# Autodesk Inventor assembly: ITEM_41115_Winkelsatz_90deg
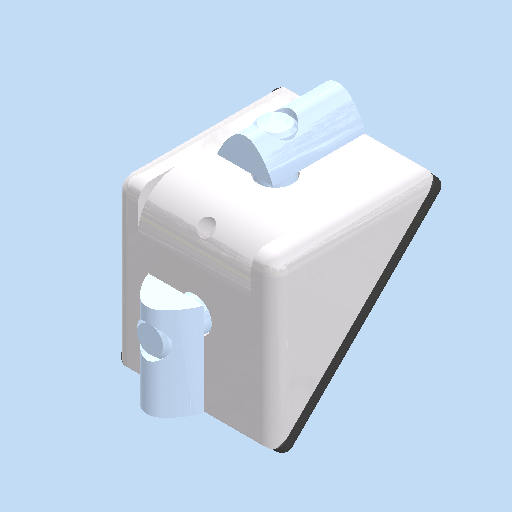
[picture p0: Inventor's stored thumbnail of the model, 512x512]
Saved by Autodesk Inventor 2023.2 (Build 272271000, 271)
## iProperties
Created: 2024-02-07
Part Number: ITEM_41115_Winkelsatz_90deg
Document SubType Name: Assembly
Designer: Nils Bade
Author: Nils Bade
## Documents named in this file (6)
- C:\Users\nilsb\Documents\Inventor\Projektarbeit-Bade\ITEM\ITEM_41115_Winkelsatz_90er.iam
- C:\Users\nilsb\Documents\Inventor\Projektarbeit-Bade\ITEM\item_winkelsatz_90er_Winkelbaustein.ipt
- C:\Users\nilsb\Documents\Inventor\Projektarbeit-Bade\ITEM\item_winkelsatz_90er_Unterlegplatte.ipt
- C:\Users\nilsb\Documents\Inventor\Projektarbeit-Bade\ITEM\item_winkelsatz_90er_Screw.ipt
- C:\Users\nilsb\Documents\Inventor\Projektarbeit-Bade\ITEM\item_winkelsatz_90er_Winkelabdeckung.ipt
- C:\Users\nilsb\Documents\Inventor\Projektarbeit-Bade\ITEM\item_winkelsatz_90er_Nutmutter.ipt
## Components (8 placed, 5 different names)
1. ITEM 4040 90er Winkelbaustein:1 — Passend:1, Passend:2, Winkel:1, Winkel:2, Passend:3, Passend:4, Passend:5, Passend:6, Passend:9, Passend:10, Passend:11, Winkel:3, Winkel:4, Passend:14, Passend:15
2. item_winkelsatz_90er_Unterlegplatte:1 — Passend:2, Winkel:1, Passend:4, Passend:8
3. item_winkelsatz_90er_Unterlegplatte:2 — Passend:1, Winkel:2, Passend:3, Passend:7
4. item_winkelsatz_90er_Screw:1 — Passend:6, Passend:8, Passend:13
5. item_winkelsatz_90er_Screw:2 — Passend:5, Passend:7, Passend:12
6. item_winkelsatz_90er_Winkelabdeckung:1 — Passend:9, Passend:10, Passend:11
7. item_winkelsatz_90er_Nutmutter:1 — Passend:12, Winkel:4, Passend:14
8. item_winkelsatz_90er_Nutmutter:2 — Passend:13, Winkel:3, Passend:15
## Relationships (19: Mate 15, Angle 4)
- Passend:1 [Mate]: ITEM 4040 90er Winkelbaustein:1 ↔ item_winkelsatz_90er_Unterlegplatte:2
- Passend:2 [Mate]: ITEM 4040 90er Winkelbaustein:1 ↔ item_winkelsatz_90er_Unterlegplatte:1
- Winkel:1 [Angle] (0 deg): ITEM 4040 90er Winkelbaustein:1 ↔ item_winkelsatz_90er_Unterlegplatte:1
- Winkel:2 [Angle] (0 deg): ITEM 4040 90er Winkelbaustein:1 ↔ item_winkelsatz_90er_Unterlegplatte:2
- Passend:3 [Mate]: ITEM 4040 90er Winkelbaustein:1 ↔ item_winkelsatz_90er_Unterlegplatte:2
- Passend:4 [Mate]: ITEM 4040 90er Winkelbaustein:1 ↔ item_winkelsatz_90er_Unterlegplatte:1
- Passend:5 [Mate]: ITEM 4040 90er Winkelbaustein:1 ↔ item_winkelsatz_90er_Screw:2
- Passend:6 [Mate]: ITEM 4040 90er Winkelbaustein:1 ↔ item_winkelsatz_90er_Screw:1
- Passend:7 [Mate]: item_winkelsatz_90er_Unterlegplatte:2 ↔ item_winkelsatz_90er_Screw:2
- Passend:8 [Mate]: item_winkelsatz_90er_Unterlegplatte:1 ↔ item_winkelsatz_90er_Screw:1
- Passend:9 [Mate]: ITEM 4040 90er Winkelbaustein:1 ↔ item_winkelsatz_90er_Winkelabdeckung:1
- Passend:10 [Mate]: ITEM 4040 90er Winkelbaustein:1 ↔ item_winkelsatz_90er_Winkelabdeckung:1
- Passend:11 [Mate]: ITEM 4040 90er Winkelbaustein:1 ↔ item_winkelsatz_90er_Winkelabdeckung:1
- Passend:12 [Mate]: item_winkelsatz_90er_Screw:2 ↔ item_winkelsatz_90er_Nutmutter:1
- Passend:13 [Mate]: item_winkelsatz_90er_Screw:1 ↔ item_winkelsatz_90er_Nutmutter:2
- Winkel:3 [Angle] (180 deg): ITEM 4040 90er Winkelbaustein:1 ↔ item_winkelsatz_90er_Nutmutter:2
- Winkel:4 [Angle] (180 deg): ITEM 4040 90er Winkelbaustein:1 ↔ item_winkelsatz_90er_Nutmutter:1
- Passend:14 [Mate] (4.5 mm): ITEM 4040 90er Winkelbaustein:1 ↔ item_winkelsatz_90er_Nutmutter:1
- Passend:15 [Mate] (4.5 mm): ITEM 4040 90er Winkelbaustein:1 ↔ item_winkelsatz_90er_Nutmutter:2
